# Autodesk Inventor assembly: Assembly_Post_v0
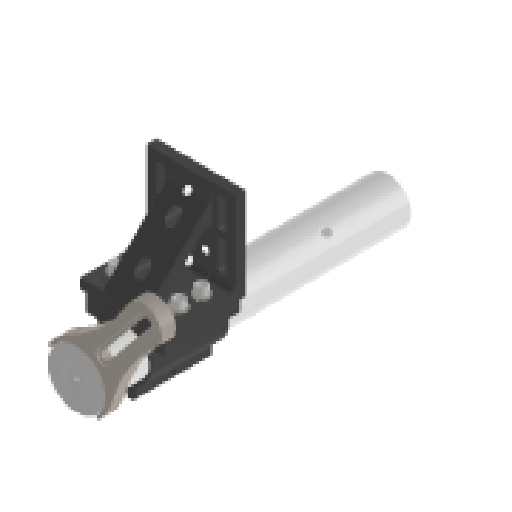
[picture p0: Inventor's stored thumbnail of the model, 512x512]
Saved by Autodesk Inventor 2024.1 (Build 281209000, 209)
## iProperties
Created: 2022-04-28
Part Number: Assembly_Post_v0
Document SubType Name: Assembly
Designer: diederichbenedict
Author: diederichbenedict
## Documents named in this file (5)
- C:\Users\diederichbenedict\Dropbox\Dokumente\Promotion\PROJECTS\SIMMO\INVENTOR\Assembly_Post_v0.iam
- C:\Users\diederichbenedict\Dropbox\Dokumente\Promotion\PROJECTS\SIMMO\INVENTOR\00_C1515_M-Step.ipt
- C:\Users\diederichbenedict\Dropbox\Dokumente\Promotion\PROJECTS\SIMMO\INVENTOR\00_PF175B-Step.ipt
- C:\Users\diederichbenedict\Dropbox\Dokumente\Promotion\PROJECTS\SIMMO\INVENTOR\00_P125_M-Step.ipt
- C:\Users\diederichbenedict\Dropbox\Dokumente\Promotion\PROJECTS\SIMMO\INVENTOR\00_PB4_M-Step.ipt
## Components (5 placed, 4 different names)
1. 00_PF175B-Step:1 — Fluchtend:1
2. 00_PB4_M-Step:1
3. 00_P125_M-Step:1
4. 00_C1515_M-Step:1 — Fluchtend:1
5. 00_P125_M-Step:2
## Relationships (5: Insert 3, Mate 1, Flush 1)
- [Insert]: 00_P125_M-Step:1 ↔ 00_P125_M-Step:2
- [Mate]: 00_C1515_M-Step:1 ↔ 00_P125_M-Step:2
- [Insert]: 00_PB4_M-Step:1 ↔ 00_P125_M-Step:1
- [Insert]: 00_PF175B-Step:1 ↔ 00_PB4_M-Step:1
- Fluchtend:1 [Flush] (110 mm): 00_PF175B-Step:1 ↔ 00_C1515_M-Step:1
